# Autodesk Inventor assembly: コックピット_1
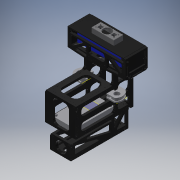
[picture p0: Inventor's stored thumbnail of the model, 180x180]
Saved by Autodesk Inventor 2018 (Build 220112000, 112)
## iProperties
Created: 2016-05-08
Part Number: コックピット_1
Document SubType Name: Assembly
Designer: hiroaki
Mass: 511.683 g
Surface Area: 1911.46 cm^2
Volume: 345.21 cm^3
Density: 1.48223 g/cm^3
Author: hiroaki
## Documents named in this file (21)
- C:\Users\taka\Documents\git\OpenPlatform\mechanism\OpenPlatform_ver3_0\上半身\コックピット\コックピット_2\コックピット_2.iam
- C:\Users\taka\Documents\git\OpenPlatform\mechanism\OpenPlatform_ver3_0\既製品\バッテリー(G6 HI-VOLTAGE 2400MAH 3S 80CMAX LIPO).ipt
- C:\Users\taka\Documents\git\OpenPlatform\mechanism\OpenPlatform_ver3_0\既製品\sw.ipt
- C:\Users\taka\Documents\git\OpenPlatform\mechanism\OpenPlatform_ver3_0\上半身\コックピット\コックピット_2\コックピット_サブフレーム_1_3.ipt
- C:\Users\taka\Documents\git\OpenPlatform\mechanism\OpenPlatform_ver3_0\上半身\コックピット\コックピット_2\コックピット_サブフレーム_1_5.ipt
- C:\Users\taka\Documents\git\OpenPlatform\mechanism\OpenPlatform_ver3_0\上半身\コックピット\コックピット_2\コックピット_サブフレーム_1_6.ipt
- C:\Users\taka\Documents\git\OpenPlatform\mechanism\OpenPlatform_ver3_0\上半身\コックピット\コックピット_2\コックピット_サブフレーム_1_7.ipt
- C:\Users\taka\Documents\git\OpenPlatform\mechanism\OpenPlatform_ver3_0\上半身\コックピット\コックピット_2\コックピット_2_メインフレーム_1.ipt
- C:\Users\taka\Documents\git\OpenPlatform\mechanism\OpenPlatform_ver3_0\上半身\コックピット\コックピット_2\コックピット_2_メインフレーム_1_MIR.ipt
- C:\Users\taka\Documents\git\OpenPlatform\mechanism\OpenPlatform_ver3_0\上半身\コックピット\コックピット_2\コックピット_2_サブフレーム_1.ipt
- C:\Users\taka\Documents\git\OpenPlatform\mechanism\OpenPlatform_ver3_0\上半身\コックピット\コックピット_2\コックピット_2_サブフレーム_2.ipt
- C:\Users\taka\Documents\git\OpenPlatform\mechanism\OpenPlatform_ver3_0\上半身\コックピット\コックピット_2\コックピット_2_サブフレーム_4.ipt
- C:\Users\taka\Documents\git\OpenPlatform\mechanism\OpenPlatform_ver3_0\上半身\コックピット\コックピット_2\コックピット_2_メインフレーム_2.ipt
- C:\Users\taka\Documents\git\OpenPlatform\mechanism\OpenPlatform_ver3_0\上半身\コックピット\コックピット_2\コックピット_2_サブフレーム_5.ipt
- C:\Users\taka\Documents\git\OpenPlatform\mechanism\OpenPlatform_ver3_0\上半身\コックピット\コックピット_2\コックピット_2_サブフレーム_6.ipt
- C:\Users\taka\Documents\git\OpenPlatform\mechanism\OpenPlatform_ver3_0\既製品\New_Accelite_Controller_Cover.ipt
- C:\Users\taka\Documents\git\OpenPlatform\mechanism\OpenPlatform_ver3_0\上半身\コックピット\コックピット_2\コックピット_サブフレーム_1_5_MIR.ipt
- C:\Users\taka\Documents\git\OpenPlatform\mechanism\OpenPlatform_ver3_0\上半身\コックピット\コックピット_2\CIT_OP_J120_Mount.ipt
- C:\Users\taka\Documents\git\OpenPlatform\mechanism\OpenPlatform_ver3_0\上半身\コックピット\コックピット_2\アンテナパーツ.ipt
- C:\Users\taka\Documents\git\OpenPlatform\mechanism\OpenPlatform_ver3_0\上半身\コックピット\コックピット_2\SwitchCov.ipt
- C:\Users\taka\Documents\git\OpenPlatform\mechanism\OpenPlatform_ver3_0\上半身\コックピット\コックピット_2\アンテナパーツ_MIR.ipt
## Components (22 placed, 20 different names)
1. バッテリー(G6 HI-VOLTAGE 2400MAH 3S 80CMAX LIPO):1 — メイト:8, メイト:12, フラッシュ:1
2. sw:1 — フラッシュ:8, フラッシュ:9, メイト:20, メイト:21, メイト:22
3. sw:2 — フラッシュ:8, フラッシュ:9, メイト:23
4. コックピット_サブフレーム_1_3:1 — メイト:12, フラッシュ:1, メイト:14, メイト:15, メイト:17, メイト:19, 挿入:40, 挿入:41, 挿入:42, 挿入:43, 挿入:60, 挿入:61
5. コックピット_サブフレーム_1_6:1 — メイト:14, メイト:15, メイト:18
6. コックピット_サブフレーム_1_5:2 — メイト:17, メイト:18, メイト:19, 挿入:23, 挿入:25
7. コックピット_サブフレーム_1_7:1 — 挿入:23, 挿入:25, メイト:49, メイト:50, メイト:51, メイト:52
8. コックピット_2_メインフレーム_1:1 — メイト:20, メイト:21, メイト:22, 挿入:40, 挿入:41, メイト:24, メイト:25, メイト:26, メイト:29, メイト:30, メイト:31, メイト:32, 挿入:48, 挿入:49, 挿入:62, 角度:1, メイト:56, メイト:57, メイト:58
9. コックピット_2_メインフレーム_1_MIR:1 — 挿入:42, 挿入:43, メイト:23, メイト:27, メイト:28, メイト:33, 挿入:50, 挿入:51, メイト:53, メイト:54, メイト:55
10. コックピット_2_サブフレーム_1:1 — メイト:24, メイト:25, メイト:26, メイト:27
11. コックピット_2_サブフレーム_2:1 — メイト:28, メイト:29, メイト:30, メイト:31, メイト:32, メイト:33, 挿入:52, 挿入:53, 挿入:54, 挿入:55, 挿入:63, 挿入:64
12. コックピット_2_サブフレーム_4:1 — 挿入:48, 挿入:49, 挿入:50, 挿入:51
13. コックピット_2_メインフレーム_2:1 — 挿入:54, 挿入:55, メイト:44, メイト:45, 挿入:56, 挿入:57
14. コックピット_2_メインフレーム_2:2 — 挿入:52, 挿入:53, メイト:43, メイト:46, 挿入:58, 挿入:59
15. コックピット_2_サブフレーム_5:1 — メイト:43, メイト:44, メイト:45, メイト:46
16. コックピット_2_サブフレーム_6:1 — 挿入:56, 挿入:57, 挿入:58, 挿入:59
17. New_Accelite_Controller_Cover:1 — メイト:49, メイト:50, メイト:51, メイト:52
18. コックピット_サブフレーム_1_5_MIR:1 — 挿入:60, 挿入:61
19. CIT_OP_J120_Mount:1 — 挿入:63, 挿入:64
20. アンテナパーツ:1 — メイト:53, メイト:54, メイト:55
21. SwitchCov:1 — 挿入:62, 角度:1
22. アンテナパーツ_MIR:1 — メイト:56, メイト:57, メイト:58
## Relationships (62: Mate 35, Insert 23, Flush 3, Angle 1)
- メイト:8 [Mate] (-52.5 mm): バッテリー(G6 HI-VOLTAGE 2400MAH 3S 80CMAX LIPO):1
- メイト:12 [Mate] (5 mm): バッテリー(G6 HI-VOLTAGE 2400MAH 3S 80CMAX LIPO):1 ↔ コックピット_サブフレーム_1_3:1
- フラッシュ:1 [Flush] (5 mm): バッテリー(G6 HI-VOLTAGE 2400MAH 3S 80CMAX LIPO):1 ↔ コックピット_サブフレーム_1_3:1
- メイト:14 [Mate] (0.05 mm): コックピット_サブフレーム_1_3:1 ↔ コックピット_サブフレーム_1_6:1
- メイト:15 [Mate]: コックピット_サブフレーム_1_3:1 ↔ コックピット_サブフレーム_1_6:1
- メイト:17 [Mate]: コックピット_サブフレーム_1_3:1 ↔ コックピット_サブフレーム_1_5:2
- メイト:18 [Mate] (0.05 mm): コックピット_サブフレーム_1_6:1 ↔ コックピット_サブフレーム_1_5:2
- メイト:19 [Mate] (0.05 mm): コックピット_サブフレーム_1_3:1 ↔ コックピット_サブフレーム_1_5:2
- 挿入:23 [Insert] (-5 mm): コックピット_サブフレーム_1_5:2 ↔ コックピット_サブフレーム_1_7:1
- 挿入:25 [Insert]: コックピット_サブフレーム_1_5:2 ↔ コックピット_サブフレーム_1_7:1
- フラッシュ:8 [Flush]: sw:1 ↔ sw:2
- フラッシュ:9 [Flush]: sw:1 ↔ sw:2
- メイト:20 [Mate]: sw:1 ↔ コックピット_2_メインフレーム_1:1
- メイト:21 [Mate] (0.55 mm): sw:1 ↔ コックピット_2_メインフレーム_1:1
- メイト:22 [Mate] (0.3 mm): sw:1 ↔ コックピット_2_メインフレーム_1:1
- 挿入:40 [Insert]: コックピット_サブフレーム_1_3:1 ↔ コックピット_2_メインフレーム_1:1
- 挿入:41 [Insert]: コックピット_サブフレーム_1_3:1 ↔ コックピット_2_メインフレーム_1:1
- 挿入:42 [Insert]: コックピット_サブフレーム_1_3:1 ↔ コックピット_2_メインフレーム_1_MIR:1
- 挿入:43 [Insert]: コックピット_サブフレーム_1_3:1 ↔ コックピット_2_メインフレーム_1_MIR:1
- メイト:23 [Mate]: sw:2 ↔ コックピット_2_メインフレーム_1_MIR:1
- メイト:24 [Mate] (0.05 mm): コックピット_2_メインフレーム_1:1 ↔ コックピット_2_サブフレーム_1:1
- メイト:25 [Mate] (0.05 mm): コックピット_2_メインフレーム_1:1 ↔ コックピット_2_サブフレーム_1:1
- メイト:26 [Mate]: コックピット_2_メインフレーム_1:1 ↔ コックピット_2_サブフレーム_1:1
- メイト:27 [Mate]: コックピット_2_メインフレーム_1_MIR:1 ↔ コックピット_2_サブフレーム_1:1
- メイト:28 [Mate]: コックピット_2_メインフレーム_1_MIR:1 ↔ コックピット_2_サブフレーム_2:1
- メイト:29 [Mate]: コックピット_2_メインフレーム_1:1 ↔ コックピット_2_サブフレーム_2:1
- メイト:30 [Mate] (0.05 mm): コックピット_2_メインフレーム_1:1 ↔ コックピット_2_サブフレーム_2:1
- メイト:31 [Mate] (0.05 mm): コックピット_2_メインフレーム_1:1 ↔ コックピット_2_サブフレーム_2:1
- メイト:32 [Mate] (0.05 mm): コックピット_2_メインフレーム_1:1 ↔ コックピット_2_サブフレーム_2:1
- メイト:33 [Mate] (0.05 mm): コックピット_2_メインフレーム_1_MIR:1 ↔ コックピット_2_サブフレーム_2:1
- 挿入:48 [Insert]: コックピット_2_メインフレーム_1:1 ↔ コックピット_2_サブフレーム_4:1
- 挿入:49 [Insert]: コックピット_2_メインフレーム_1:1 ↔ コックピット_2_サブフレーム_4:1
- 挿入:50 [Insert]: コックピット_2_メインフレーム_1_MIR:1 ↔ コックピット_2_サブフレーム_4:1
- 挿入:51 [Insert]: コックピット_2_メインフレーム_1_MIR:1 ↔ コックピット_2_サブフレーム_4:1
- 挿入:52 [Insert]: コックピット_2_サブフレーム_2:1 ↔ コックピット_2_メインフレーム_2:2
- 挿入:53 [Insert]: コックピット_2_サブフレーム_2:1 ↔ コックピット_2_メインフレーム_2:2
- 挿入:54 [Insert]: コックピット_2_サブフレーム_2:1 ↔ コックピット_2_メインフレーム_2:1
- 挿入:55 [Insert]: コックピット_2_サブフレーム_2:1 ↔ コックピット_2_メインフレーム_2:1
- メイト:43 [Mate] (0.05 mm): コックピット_2_メインフレーム_2:2 ↔ コックピット_2_サブフレーム_5:1
- メイト:44 [Mate] (0.05 mm): コックピット_2_メインフレーム_2:1 ↔ コックピット_2_サブフレーム_5:1
- メイト:45 [Mate]: コックピット_2_メインフレーム_2:1 ↔ コックピット_2_サブフレーム_5:1
- メイト:46 [Mate]: コックピット_2_メインフレーム_2:2 ↔ コックピット_2_サブフレーム_5:1
- 挿入:56 [Insert]: コックピット_2_メインフレーム_2:1 ↔ コックピット_2_サブフレーム_6:1
- 挿入:57 [Insert]: コックピット_2_メインフレーム_2:1 ↔ コックピット_2_サブフレーム_6:1
- 挿入:58 [Insert]: コックピット_2_メインフレーム_2:2 ↔ コックピット_2_サブフレーム_6:1
- 挿入:59 [Insert]: コックピット_2_メインフレーム_2:2 ↔ コックピット_2_サブフレーム_6:1
- メイト:49 [Mate]: コックピット_サブフレーム_1_7:1 ↔ New_Accelite_Controller_Cover:1
- メイト:50 [Mate]: コックピット_サブフレーム_1_7:1 ↔ New_Accelite_Controller_Cover:1
- メイト:51 [Mate]: コックピット_サブフレーム_1_7:1 ↔ New_Accelite_Controller_Cover:1
- メイト:52 [Mate]: コックピット_サブフレーム_1_7:1 ↔ New_Accelite_Controller_Cover:1
- 挿入:60 [Insert]: コックピット_サブフレーム_1_3:1 ↔ コックピット_サブフレーム_1_5_MIR:1
- 挿入:61 [Insert]: コックピット_サブフレーム_1_3:1 ↔ コックピット_サブフレーム_1_5_MIR:1
- 挿入:62 [Insert]: コックピット_2_メインフレーム_1:1 ↔ SwitchCov:1
- 挿入:63 [Insert]: コックピット_2_サブフレーム_2:1 ↔ CIT_OP_J120_Mount:1
- 角度:1 [Angle] (180 deg): コックピット_2_メインフレーム_1:1 ↔ SwitchCov:1
- 挿入:64 [Insert]: コックピット_2_サブフレーム_2:1 ↔ CIT_OP_J120_Mount:1
- メイト:53 [Mate]: コックピット_2_メインフレーム_1_MIR:1 ↔ アンテナパーツ:1
- メイト:54 [Mate]: コックピット_2_メインフレーム_1_MIR:1 ↔ アンテナパーツ:1
- メイト:55 [Mate] (4 mm): コックピット_2_メインフレーム_1_MIR:1 ↔ アンテナパーツ:1
- メイト:56 [Mate]: コックピット_2_メインフレーム_1:1 ↔ アンテナパーツ_MIR:1
- メイト:57 [Mate]: コックピット_2_メインフレーム_1:1 ↔ アンテナパーツ_MIR:1
- メイト:58 [Mate] (4 mm): コックピット_2_メインフレーム_1:1 ↔ アンテナパーツ_MIR:1
